# Autodesk Inventor assembly: ASY GBK 1320 long wall shield 5
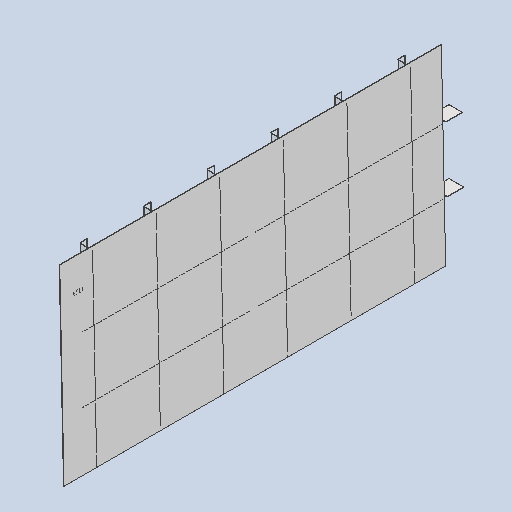
[picture p0: Inventor's stored thumbnail of the model, 512x512]
Saved by Autodesk Inventor 2026 (Build 300175000, 175)
## iProperties
Created: 2026-05-07
Part Number: ASY GBK 1320 long wall shield 5
Document SubType Name: Assembly
Designer: pokla
Mass: 215512 g
Surface Area: 139105 cm^2
Volume: 27453.8 cm^3
Density: 7.85 g/cm^3
Stock Number: 1321
Author: admin
## Documents named in this file (6)
- C:\Users\pokla\Documents\Inventor\GBK-Gubkinskiy\ASY GBK 1320 long wall shield 5.iam
- C:\Users\pokla\Documents\Inventor\GBK-Gubkinskiy\GBK 0101 main rib.ipt
- C:\Users\pokla\Documents\Inventor\GBK-Gubkinskiy\GBK 0302 stringer 7.ipt
- C:\Users\pokla\Documents\Inventor\GBK-Gubkinskiy\GBK 0303 stringer 8.ipt
- C:\Users\pokla\Documents\Inventor\GBK-Gubkinskiy\GBK 0301 third rib.ipt
- C:\Users\pokla\Documents\Inventor\GBK-Gubkinskiy\GBK 1325 shield 1.2.ipt
## Components (11 placed, 4 different names)
1. GBK 0302 stringer 7.ipt:1 — Жесткий:4
2. GBK 0303 stringer 8.ipt:1 — Жесткий:3, Совмещение:2, Заподлицо:2
3. GBK 0303 stringer 8.ipt:2 — Жесткий:3
4. GBK 0302 stringer 7.ipt:2 — Жесткий:4
5. GBK 1325 shield 1.2:1 — Совмещение:3, Заподлицо:1, Совмещение:4, Заподлицо:2
6. GBK 0301 third rib.ipt:1 — Совмещение:1, Совмещение:3
7. GBK 0301 third rib.ipt:2
8. GBK 0301 third rib.ipt:3
9. GBK 0301 third rib.ipt:4
10. GBK 0301 third rib.ipt:5
11. GBK 0301 third rib.ipt:6
## Component patterns: (6 elements, first: GBK 0301 third rib.ipt:1)
## Relationships (10: WeldJoint 4, Mate 4, Flush 2)
- [WeldJoint] (4 mm): GBK 0302 stringer 7.ipt:1 ↔ GBK 0301 third rib.ipt:1
- [WeldJoint] (4 mm): GBK 0303 stringer 8.ipt:1 ↔ GBK 0301 third rib.ipt:1
- Жесткий:3 [WeldJoint] (1 mm): GBK 0303 stringer 8.ipt:1 ↔ GBK 0303 stringer 8.ipt:2
- Жесткий:4 [WeldJoint] (1 mm): GBK 0302 stringer 7.ipt:1 ↔ GBK 0302 stringer 7.ipt:2
- Совмещение:1 [Mate]: GBK 0301 third rib.ipt:1
- Совмещение:2 [Mate]: GBK 0303 stringer 8.ipt:1
- Совмещение:3 [Mate]: GBK 1325 shield 1.2:1 ↔ GBK 0301 third rib.ipt:1
- Заподлицо:1 [Flush]: GBK 1325 shield 1.2:1
- Совмещение:4 [Mate]: GBK 1325 shield 1.2:1
- Заподлицо:2 [Flush] (155 mm): GBK 0303 stringer 8.ipt:1 ↔ GBK 1325 shield 1.2:1
## Named parameters: Шаг_шпангоутов = 496.66667 mm
